# Autodesk Inventor assembly: output_assembly
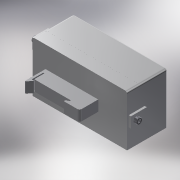
[picture p0: Inventor's stored thumbnail of the model, 180x180]
Saved by Autodesk Inventor 2019 (Build 230136000, 136)
## iProperties
Created: 2020-05-12
Part Number: output_assembly
Document SubType Name: Assembly
Designer: Mateusz
Author: Mateusz
## Documents named in this file (6)
- D:\Projekty\Azure Sphere IoT Controller\Addons\Output\case\output_assembly.iam
- D:\Projekty\Azure Sphere IoT Controller\Addons\Output\case\output_board.ipt
- D:\Projekty\Azure Sphere IoT Controller\Addons\Output\case\bottom.ipt
- D:\Projekty\Azure Sphere IoT Controller\Addons\Output\case\top.ipt
- D:\Projekty\Azure Sphere IoT Controller\Addons\Output\case\SHCS M3-20.ipt
- D:\Projekty\Azure Sphere IoT Controller\Addons\Output\case\DIN_mount.ipt
## Components (7 placed, 5 different names)
1. output_board:1 — Mate:1, Mate:2, Mate:3
2. bottom:1 — Mate:1, Mate:2, Mate:3, Flush:1, Mate:4, Flush:2, Mate:11, Mate:12, Mate:13
3. top:1 — Flush:1, Mate:4, Flush:2, Mate:5, Mate:6, Mate:7, Mate:8, Mate:9, Mate:10
4. SHCS M3-20:1 — Mate:5, Mate:10
5. SHCS M3-20:2 — Mate:6, Mate:9
6. SHCS M3-20:3 — Mate:7, Mate:8
7. DIN_mount:1 — Mate:11, Mate:12, Mate:13
## Relationships (15: Mate 13, Flush 2)
- Mate:1: output_board:1 ↔ bottom:1
- Mate:2: output_board:1 ↔ bottom:1
- Mate:3 (0.5 mm): output_board:1 ↔ bottom:1
- Flush:1: bottom:1 ↔ top:1
- Mate:4: bottom:1 ↔ top:1
- Flush:2: bottom:1 ↔ top:1
- Mate:5: top:1 ↔ SHCS M3-20:1
- Mate:6: top:1 ↔ SHCS M3-20:2
- Mate:7: top:1 ↔ SHCS M3-20:3
- Mate:8: top:1 ↔ SHCS M3-20:3
- Mate:9: top:1 ↔ SHCS M3-20:2
- Mate:10: top:1 ↔ SHCS M3-20:1
- Mate:11: bottom:1 ↔ DIN_mount:1
- Mate:12: bottom:1 ↔ DIN_mount:1
- Mate:13: bottom:1 ↔ DIN_mount:1
